# Autodesk Inventor assembly: Magnet
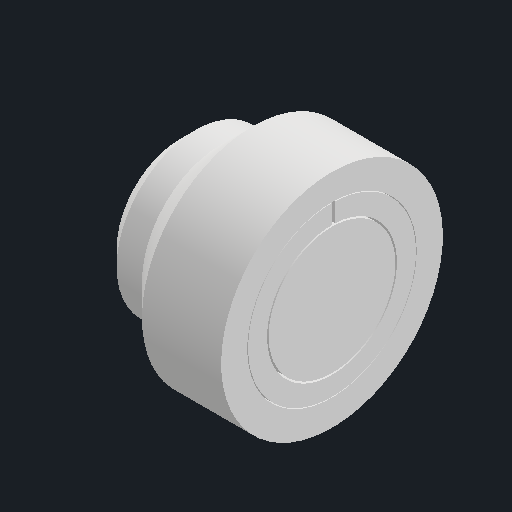
[picture p0: Inventor's stored thumbnail of the model, 512x512]
Saved by Autodesk Inventor 2022 (Build 260153000, 153)
## iProperties
Created: 2022-03-29
Part Number: Magnet
Document SubType Name: Assembly
Designer: neko2
Author: neko2
## Documents named in this file (4)
- C:\Users\neko2\OneDrive\reRo\MicroMouse\SaponseEx\CAD\Magnet.iam
- C:\Users\neko2\OneDrive\reRo\MicroMouse\SaponseEx\CAD\Magnet.ipt
- C:\Users\neko2\OneDrive\reRo\MicroMouse\SaponseEx\CAD\Spacer.ipt
- C:\Users\neko2\OneDrive\reRo\MicroMouse\SaponseEx\CAD\MagnetMounter.ipt
## Components (3 placed, 3 different names)
1. Magnet:1 — メイト:2, フラッシュ:1
2. Spacer:1 — メイト:1, メイト:2, フラッシュ:1, フラッシュ:2
3. MagnetMounter:1 — メイト:1, フラッシュ:2
## Relationships (4: Mate 2, Flush 2)
- メイト:1 [Mate]: Spacer:1 ↔ MagnetMounter:1
- メイト:2 [Mate]: Magnet:1 ↔ Spacer:1
- フラッシュ:1 [Flush]: Magnet:1 ↔ Spacer:1
- フラッシュ:2 [Flush]: Spacer:1 ↔ MagnetMounter:1
